# Autodesk Inventor assembly: A Drive
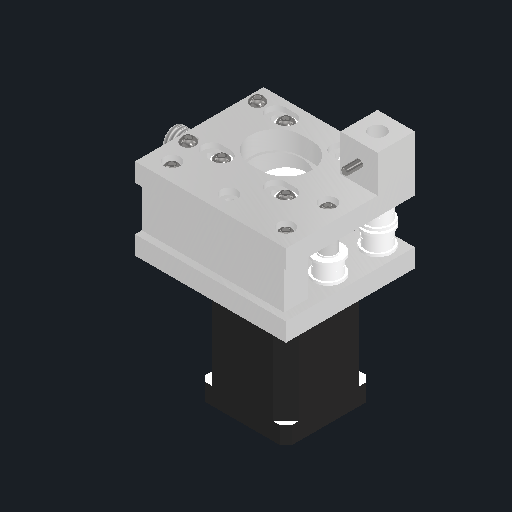
[picture p0: Inventor's stored thumbnail of the model, 512x512]
Saved by Autodesk Inventor 2025.1 (Build 291241020, 241B)
## iProperties
Created: 2025-05-09
Part Number: A Drive
Document SubType Name: Assembly
Designer: AdminForWorker
Title: A Drive
Author: AdminForWorker
## Documents named in this file (4)
- C:\Users\Joshua Eah\Documents\Voron 0.2\CAD\Master Assembly\A Drive.iam
- C:\Users\Joshua Eah\Documents\Voron 0.2\CAD\Master Assembly\Motor Assembly.iam
- C:\Users\Joshua Eah\Documents\Voron 0.2\CAD\Master Assembly\Hardware\Hardware Assemblies\Hardware (7).iam
- C:\Users\Joshua Eah\Documents\Voron 0.2\CAD\Machined Parts\AB Drives\A Drive\A Drive Assembly.iam
## Components (3 placed, 3 different names)
1. Motor Assembly:1 [sub-assembly]
2. A Drive Assembly:1 [sub-assembly] — Insert:1, Insert:2
3. Hardware (7):1 [sub-assembly] — Insert:1, Insert:2
## Relationships (2: Insert 2)
- Insert:1: A Drive Assembly:1 ↔ Hardware (7):1
- Insert:2: A Drive Assembly:1 ↔ Hardware (7):1
